# Autodesk Inventor assembly: custom_asembly
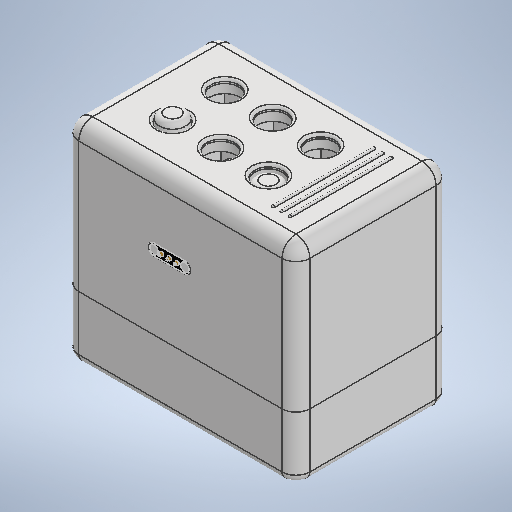
[picture p0: Inventor's stored thumbnail of the model, 512x512]
Saved by Autodesk Inventor 2025.1 (Build 291241000, 241)
## iProperties
Created: 2025-02-27
Part Number: custom_asembly
Document SubType Name: Assembly
Designer: santiago
Author: santiago
## Documents named in this file (17)
- C:\Users\santiago\Documents\Tesis\3d models\scaled\CUSTOM\custom_asembly.iam
- C:\Users\santiago\Documents\Tesis\3d models\scaled\CUSTOM\Part3.ipt
- C:\Users\santiago\Documents\Tesis\3d models\scaled\CUSTOM\Part4.ipt
- C:\Users\santiago\Documents\Tesis\3d models\scaled\CUSTOM\Assembly1.iam
- C:\Users\santiago\Documents\Tesis\3d models\scaled\Electromagnet.ipt
- C:\Users\santiago\Documents\Tesis\3d models\scaled\CUSTOM\Part5.ipt
- C:\Users\santiago\Documents\Tesis\3d models\Top_layer.iam
- C:\Users\santiago\Documents\Tesis\3d models\Bottom_layer.iam
- C:\Users\santiago\Documents\Tesis\3d models\conn_enclosure.ipt
- C:\Users\santiago\Documents\Tesis\3d models\conn\shell_top.ipt
- C:\Users\santiago\Documents\Tesis\3d models\conn\shell_bttm.ipt
- C:\Users\santiago\Documents\Tesis\3d models\conn\2_pin_ear_female.ipt
- C:\Users\santiago\Documents\Tesis\3d models\conn\3_pin_ear_female.ipt
- C:\Users\santiago\Documents\Tesis\3d models\conn\3_pin_no_ear_male.ipt
- C:\Users\santiago\Documents\Chamba\friction experiment\experiment_thread_insert.ipt
- C:\Users\santiago\Documents\Tesis\3d models\conn\M3 x 10.ipt
- C:\Users\santiago\Documents\Tesis\3d models\conn\M3 x 16.ipt
## Components (31 placed, 16 different names)
1. Part3:1 — Flush:1, Flush:2, Mate:1, Flush:3, Flush:4, Mate:2, Mate:3, Flush:5, Flush:8, Flush:7, Mate:4, Mate:5, Mate:6, Insert:1, Flush:9, Mate:10, Mate:11, Mate:12, Mate:13, Mate:15, Mate:16, Mate:23, Mate:24
2. Part4:1 — Flush:1, Mate:8, Mate:9, Flush:9, Mate:10, Flush:10, Mate:25, Mate:26
3. Assembly1:1 [sub-assembly] — Flush:2, Mate:1
4. Assembly1:2 [sub-assembly] — Flush:3, Mate:2
5. Assembly1:3 [sub-assembly] — Flush:4, Mate:3
6. Assembly1:4 [sub-assembly] — Flush:5, Mate:4
7. Assembly1:5 [sub-assembly] — Flush:7, Mate:6
8. Assembly1:6 [sub-assembly] — Flush:8, Mate:5
9. Electromagnet:1 — Insert:1
10. Part5:1 — Mate:8
11. Part5:2 — Mate:9
12. Top_layer:1 [sub-assembly] — Mate:11, Mate:12, Mate:13, Mate:14
13. Bottom_layer:1 [sub-assembly] — Mate:14, Mate:15, Mate:16
14. conn_enclosure:1 — Mate:23, Mate:24, Insert:5
15. shell_top:1 — Flush:10, Flush:11, Flush:12, Mate:17, Mate:18, Flush:13, Mate:19, Mate:20, Mate:25, Mate:26, Mate:27, Flush:15, Insert:2, Insert:3
16. shell_bttm:1 — Flush:11, Flush:14, Mate:21, Mate:22, Mate:27, Flush:15, Insert:4
17. 3_pin_ear_female:1 — Flush:13, Mate:19, Mate:20
18. 3_pin_no_ear_male:1 — Flush:12, Mate:17, Mate:18
19. 2_pin_ear_female:1 — Flush:14, Mate:21, Mate:22
20. experiment_thread_insert:5 — Insert:2
21. experiment_thread_insert:7
22. experiment_thread_insert:8
23. experiment_thread_insert:9
24. experiment_thread_insert:6 — Insert:3
25. experiment_thread_insert:10
26. M3 x 16:1 — Insert:4
27. M3 x 16:2
28. M3 x 16:3
29. M3 x 16:4
30. M3 x 10:1 — Insert:5
31. M3 x 10:2
## Component patterns: (4 elements, first: experiment_thread_insert:5), (2 elements, first: experiment_thread_insert:6), (4 elements, first: M3 x 16:1), (2 elements, first: M3 x 10:1)
## Relationships (45: Mate 26, Flush 14, Insert 5)
- Flush:1: Part3:1 ↔ Part4:1
- Flush:2: Part3:1 ↔ Assembly1:1
- Mate:1: Part3:1 ↔ Assembly1:1
- Flush:3: Part3:1 ↔ Assembly1:2
- Flush:4: Part3:1 ↔ Assembly1:3
- Mate:2: Part3:1 ↔ Assembly1:2
- Mate:3: Part3:1 ↔ Assembly1:3
- Flush:5: Part3:1 ↔ Assembly1:4
- Flush:8: Part3:1 ↔ Assembly1:6
- Flush:7: Part3:1 ↔ Assembly1:5
- Mate:4: Part3:1 ↔ Assembly1:4
- Mate:5: Part3:1 ↔ Assembly1:6
- Mate:6: Part3:1 ↔ Assembly1:5
- Insert:1: Part3:1 ↔ Electromagnet:1
- Mate:8: Part4:1 ↔ Part5:1
- Mate:9: Part4:1 ↔ Part5:2
- Flush:9: Part3:1 ↔ Part4:1
- Mate:10: Part3:1 ↔ Part4:1
- Mate:11: Part3:1 ↔ Top_layer:1
- Mate:12: Part3:1 ↔ Top_layer:1
- Mate:13: Part3:1 ↔ Top_layer:1
- Mate:14: Top_layer:1 ↔ Bottom_layer:1
- Mate:15: Part3:1 ↔ Bottom_layer:1
- Mate:16: Part3:1 ↔ Bottom_layer:1
- Flush:10: Part4:1 ↔ shell_top:1
- Flush:11: shell_top:1 ↔ shell_bttm:1
- Flush:12: shell_top:1 ↔ 3_pin_no_ear_male:1
- Mate:17: shell_top:1 ↔ 3_pin_no_ear_male:1
- Mate:18: shell_top:1 ↔ 3_pin_no_ear_male:1
- Flush:13: shell_top:1 ↔ 3_pin_ear_female:1
- Mate:19: shell_top:1 ↔ 3_pin_ear_female:1
- Mate:20: shell_top:1 ↔ 3_pin_ear_female:1
- Flush:14: shell_bttm:1 ↔ 2_pin_ear_female:1
- Mate:21: shell_bttm:1 ↔ 2_pin_ear_female:1
- Mate:22: shell_bttm:1 ↔ 2_pin_ear_female:1
- Mate:23: Part3:1 ↔ conn_enclosure:1
- Mate:24: Part3:1 ↔ conn_enclosure:1
- Mate:25: Part4:1 ↔ shell_top:1
- Mate:26: Part4:1 ↔ shell_top:1
- Mate:27: shell_top:1 ↔ shell_bttm:1
- Flush:15: shell_top:1 ↔ shell_bttm:1
- Insert:2 (-0.01 mm): shell_top:1 ↔ experiment_thread_insert:5
- Insert:3 (-0.01 mm): shell_top:1 ↔ experiment_thread_insert:6
- Insert:4: shell_bttm:1 ↔ M3 x 16:1
- Insert:5: conn_enclosure:1 ↔ M3 x 10:1
## Named parameters: row = 72.5 mm, column = 60.8 mm
